# Autodesk Inventor assembly: CAR_047_FullSweeperAssembly
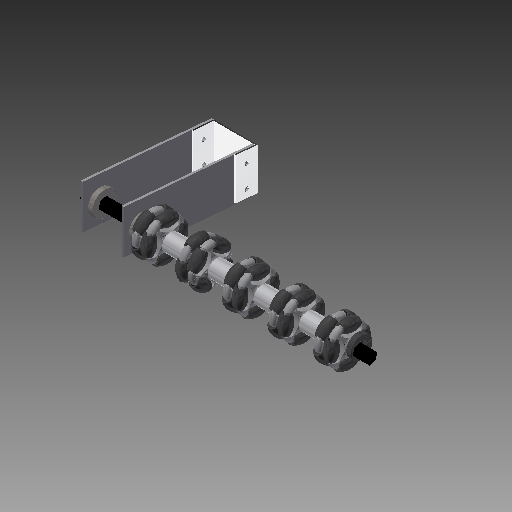
[picture p0: Inventor's stored thumbnail of the model, 512x512]
Saved by Autodesk Inventor 2018.3 (Build 223284000, 284)
## iProperties
Created: 2020-02-16
Part Number: CAR_047_FullSweeperAssembly
Document SubType Name: Assembly
Designer: jd2
Author: jd2
## Documents named in this file (6)
- C:\Users\22barlalex\Documents\GrabCAD\Infinite Recharge 2020\Build season\CAR_052_FullSweeperAssembly.iam
- C:\Users\22barlalex\Documents\GrabCAD\Infinite Recharge 2020\Build season\CAR_049_SweeperBarMount.ipt
- C:\Users\22barlalex\Documents\GrabCAD\Infinite Recharge 2020\Build season\CAR_050_Sweeper Bar arms.ipt
- C:\Users\22barlalex\Documents\GrabCAD\Infinite Recharge 2020\Build season\CAR_051_HalfInchHexBearing.ipt
- C:\Users\22barlalex\Documents\GrabCAD\Infinite Recharge 2020\Build season\CAR_034_SweeperBarAssembly.iam
- C:\Users\22barlalex\Documents\GrabCAD\Infinite Recharge 2020\Build season\CAR_053_HalfInchHexCollar.ipt
## Components (8 placed, 5 different names)
1. CAR_049_SweeperBarMount:1 — Mate:9, Flush:2, Flush:3, Mate:10, Flush:4, Mate:11
2. CAR_050_Sweeper Bar arms:1 — Mate:3, Insert:1, Mate:8, Mate:9, Flush:2, Flush:3
3. CAR_051_HalfInchHexBearing:1 — Mate:3, Mate:4, Mate:5, Insert:1, Mate:8
4. CAR_034_SweeperBarAssembly:1 [sub-assembly] — Mate:4, Mate:5, Mate:12, Flush:5, Mate:13, Mate:14, Flush:6
5. CAR_050_Sweeper Bar arms:2 — Insert:2, Mate:10, Flush:4, Mate:11
6. CAR_051_HalfInchHexBearing:2 — Insert:2
7. CAR_053_HalfInchHexCollar:1 — Mate:12, Flush:5
8. CAR_053_HalfInchHexCollar:2 — Mate:13, Mate:14, Flush:6
## Relationships (17: Mate 10, Flush 5, Insert 2)
- Mate:3: CAR_050_Sweeper Bar arms:1 ↔ CAR_051_HalfInchHexBearing:1
- Mate:4: CAR_051_HalfInchHexBearing:1 ↔ CAR_034_SweeperBarAssembly:1
- Mate:5: CAR_051_HalfInchHexBearing:1 ↔ CAR_034_SweeperBarAssembly:1
- Insert:1: CAR_050_Sweeper Bar arms:1 ↔ CAR_051_HalfInchHexBearing:1
- Mate:8: CAR_050_Sweeper Bar arms:1 ↔ CAR_051_HalfInchHexBearing:1
- Mate:9: CAR_049_SweeperBarMount:1 ↔ CAR_050_Sweeper Bar arms:1
- Flush:2: CAR_049_SweeperBarMount:1 ↔ CAR_050_Sweeper Bar arms:1
- Flush:3: CAR_049_SweeperBarMount:1 ↔ CAR_050_Sweeper Bar arms:1
- Insert:2: CAR_050_Sweeper Bar arms:2 ↔ CAR_051_HalfInchHexBearing:2
- Mate:10: CAR_049_SweeperBarMount:1 ↔ CAR_050_Sweeper Bar arms:2
- Flush:4: CAR_049_SweeperBarMount:1 ↔ CAR_050_Sweeper Bar arms:2
- Mate:11: CAR_049_SweeperBarMount:1 ↔ CAR_050_Sweeper Bar arms:2
- Mate:12: CAR_034_SweeperBarAssembly:1 ↔ CAR_053_HalfInchHexCollar:1
- Flush:5 (14.224 mm): CAR_034_SweeperBarAssembly:1 ↔ CAR_053_HalfInchHexCollar:1
- Mate:13: CAR_034_SweeperBarAssembly:1 ↔ CAR_053_HalfInchHexCollar:2
- Mate:14: CAR_034_SweeperBarAssembly:1 ↔ CAR_053_HalfInchHexCollar:2
- Flush:6 (6.096 mm): CAR_034_SweeperBarAssembly:1 ↔ CAR_053_HalfInchHexCollar:2
